# Autodesk Inventor assembly: 1590E
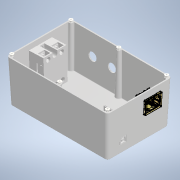
[picture p0: Inventor's stored thumbnail of the model, 180x180]
Saved by Autodesk Inventor 2020.2 (Build 242310000, 310)
## iProperties
Created: 2015-07-13
Part Number: 1590E
Document SubType Name: Assembly
Designer: elmar
Sending System: Autodesk Inventor 2015
Preprocessor: ST-DEVELOPER v15.6
Title: E:\Eng\Customer Service\Drawings\1590\STEP\1590E.stp
Author: mbeerman
## Documents named in this file (7)
- C:\Users\elmar\OneDrive\Inventor\LEGEND\PressureBuildingHeaterController\1590E.iam
- C:\Users\elmar\OneDrive\Inventor\LEGEND\PressureBuildingHeaterController\1590E BOX.ipt
- C:\Users\elmar\OneDrive\Inventor\LEGEND\PressureBuildingHeaterController\1590D-DD-E LID.ipt
- C:\Users\elmar\OneDrive\Inventor\LEGEND\PressureBuildingHeaterController\SC530 (screw #6-32X 1_2'' FH).ipt
- C:\Users\elmar\OneDrive\Inventor\LEGEND\PressureBuildingHeaterController\701wx202.iam
- C:\Users\elmar\OneDrive\Inventor\LEGEND\PressureBuildingHeaterController\G3NA_220B.ipt
- C:\Users\elmar\OneDrive\Inventor\LEGEND\PressureBuildingHeaterController\arduino uno.ipt
## Components (11 placed, 6 different names)
1. 1590E BOX:1 — Flush:1, Mate:1, Mate:2, Mate:3, Mate:4, Mate:6, Mate:7, Mate:8
2. 1590D-DD-E LID:1
3. SC530 (screw #6-32X 1_2'' FH):5
4. SC530 (screw #6-32X 1_2'' FH):6
5. SC530 (screw #6-32X 1_2'' FH):1
6. SC530 (screw #6-32X 1_2'' FH):2
7. SC530 (screw #6-32X 1_2'' FH):3
8. SC530 (screw #6-32X 1_2'' FH):4
9. 701wx202:1 [sub-assembly] — Flush:1, Mate:1, Mate:2
10. G3NA_220B:1 — Mate:3, Mate:4, Mate:5
11. arduino uno:1 — Mate:6, Mate:7, Mate:8
## Relationships (9: Mate 8, Flush 1)
- Flush:1: 1590E BOX:1 ↔ 701wx202:1
- Mate:1 (40 mm): 1590E BOX:1 ↔ 701wx202:1
- Mate:2 (15 mm): 1590E BOX:1 ↔ 701wx202:1
- Mate:3 (0.5 mm): 1590E BOX:1 ↔ G3NA_220B:1
- Mate:4 (-8.75 mm): 1590E BOX:1 ↔ G3NA_220B:1
- Mate:5: G3NA_220B:1
- Mate:6 (10 mm): 1590E BOX:1 ↔ arduino uno:1
- Mate:7: 1590E BOX:1 ↔ arduino uno:1
- Mate:8 (10 mm): 1590E BOX:1 ↔ arduino uno:1
